# Autodesk Inventor assembly: Prototype Assembly
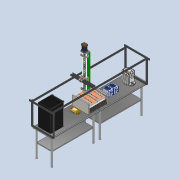
[picture p0: Inventor's stored thumbnail of the model, 180x180]
Saved by Autodesk Inventor 2022 (Build 260153000, 153)
## iProperties
Created: 2021-10-10
Part Number: Prototype Assembly
Document SubType Name: Assembly
Designer: Coy
Author: Coy
## Documents named in this file (14)
- H:\3D Files\Project 3D Models\Breakfast Maker 2000\Assemblys\Prototype Assembly.iam
- H:\3D Files\Project 3D Models\Stock Parts\Workshop\60in Kitchen Prep Table.ipt
- H:\3D Files\Project 3D Models\Stock Parts\Aluminum Extrusion\2040\2040x700 silver profile.ipt
- H:\3D Files\Project 3D Models\Stock Parts\Aluminum Extrusion\2040\2040x1000 silver profile.ipt
- H:\3D Files\Project 3D Models\Stock Parts\Workshop\27in Tall Mini Fridge.ipt
- H:\3D Files\Project 3D Models\Stock Parts\Aluminum Extrusion\2040\2040x800 silver profile.ipt
- H:\3D Files\Project 3D Models\Stock Parts\Workshop\Kureig Assembly.iam
- H:\3D Files\Project 3D Models\Stock Parts\Workshop\Roller hot dogs.ipt
- H:\3D Files\Project 3D Models\Stock Parts\Workshop\TOASTER_BY_TRISTAN_CANNAN.iam
- H:\3D Files\Project 3D Models\Stock Parts\Workshop\waffle_maker.ipt
- H:\3D Files\Project 3D Models\Stock Parts\Linear Actuators\Ball Screw Linear Actuator.iam
- H:\3D Files\Project 3D Models\Stock Parts\Linear Actuators\MGN12C Linear Rail.iam
- H:\3D Files\Downloaded 3D Files\GrabCad Downloads\hiwin-mgn-series-full-2.snapshot.14\PRODUCT_NAME_10.ipt
- H:\3D Files\Project 3D Models\Breakfast Maker 2000\Generic 4x3in Steel Square Tubing.ipt
## Components (40 placed, 13 different names)
1. 60in Kitchen Prep Table:1 — Flush:1, Mate:1, Flush:2, Mate:3, Mate:25, Mate:26, Mate:27, Mate:28
2. 60in Kitchen Prep Table:2 — Flush:1, Mate:1, Flush:2, Mate:2, Flush:3, Flush:5, Mate:20, Flush:36, Mate:24
3. 2040x700 silver profile:1 — Mate:2, Flush:3, Flush:4, Flush:5, Flush:7, Flush:9, Mate:16, Flush:30, Mate:17, Flush:31, Mate:21
4. 2040x700 silver profile:2 — Mate:3, Flush:4, Flush:11, Flush:13, Mate:14, Mate:15, Flush:28, Flush:29
5. 2040x700 silver profile:3 — Flush:13, Flush:27, Mate:14, Flush:28
6. 2040x700 silver profile:4 — Flush:11, Mate:15, Flush:29, Mate:23
7. 2040x700 silver profile:5 — Flush:9, Mate:9, Flush:17, Flush:18, Mate:17, Flush:31
8. 2040x700 silver profile:6 — Flush:7, Mate:8, Flush:15, Flush:16, Mate:16, Flush:30, Mate:22, Flush:38, Flush:39
9. 2040x1000 silver profile:1 — Mate:12, Flush:23, Flush:24
10. 2040x1000 silver profile:2 — Mate:11, Flush:21, Flush:22, Mate:12, Flush:23, Flush:24
11. 2040x1000 silver profile:3 — Mate:8, Flush:15, Flush:16, Mate:10, Flush:19, Flush:20, Mate:29, Flush:42
12. 2040x1000 silver profile:4 — Mate:9, Flush:17, Flush:18, Mate:11, Flush:21, Flush:22
13. 2040x1000 silver profile:5 — Mate:10, Flush:19, Flush:20, Mate:13, Flush:25, Flush:26, Mate:30
14. 2040x1000 silver profile:6 — Mate:13, Flush:25, Flush:26, Flush:27, Flush:41
15. 27in Tall Mini Fridge:1 — Mate:20, Mate:21, Flush:36
16. 2040x800 silver profile:1 — Mate:22, Flush:38, Flush:39, Flush:40
17. 2040x800 silver profile:2 — Mate:23, Flush:40, Flush:41
18. Kureig Assembly:1 [sub-assembly] — Mate:26
19. Roller hot dogs:1 — Mate:25
20. TOASTER_BY_TRISTAN_CANNAN:1 [sub-assembly] — Mate:27
21. waffle_maker:1 — Mate:24
22. TOASTER_BY_TRISTAN_CANNAN:2 [sub-assembly] — Mate:28
23. 2040x700 silver profile:7 — Mate:30, Flush:43, Mate:31, Mate:33, Flush:46, Flush:58
24. 2040x700 silver profile:8 — Mate:29, Flush:42, Flush:43, Mate:31, Mate:32, Flush:45, Mate:34, Flush:47, Mate:35
25. Ball Screw Linear Actuator:1 [sub-assembly] — Mate:49, Flush:72
26. MGN12C Linear Rail:1 [sub-assembly] — Mate:32, Flush:44, Flush:45, Flush:48, Mate:36, Flush:49, Mate:38, Flush:50, Flush:51, Mate:47, Mate:48
27. MGN12C Linear Rail:2 [sub-assembly] — Mate:33, Flush:44, Flush:46, Flush:59, Flush:61, Flush:62, Mate:43, Flush:63, Flush:64
28. PRODUCT_NAME_10:1 — Mate:38, Flush:50, Flush:51, Mate:39, Flush:52, Flush:53
29. PRODUCT_NAME_10:2 — Flush:58, Flush:59, Flush:60, Mate:42
30. PRODUCT_NAME_10:3 — Mate:43, Flush:63, Flush:64, Mate:44, Flush:65, Flush:66
31. PRODUCT_NAME_10:4 — Mate:44, Flush:65, Flush:66, Mate:45, Flush:67, Flush:68
32. PRODUCT_NAME_10:5 — Mate:40, Flush:54, Flush:55, Mate:41, Flush:56, Flush:57
33. PRODUCT_NAME_10:6 — Mate:35, Mate:36, Mate:37, Flush:49
34. PRODUCT_NAME_10:7 — Mate:39, Flush:52, Flush:53, Mate:40, Flush:54, Flush:55
35. PRODUCT_NAME_10:8 — Mate:42, Flush:61, Flush:62
36. PRODUCT_NAME_10:9 — Mate:45, Flush:67, Flush:68, Mate:46, Flush:69, Flush:70
37. PRODUCT_NAME_10:10 — Mate:46, Flush:69, Flush:70
38. PRODUCT_NAME_10:11 — Mate:41, Flush:56, Flush:57
39. PRODUCT_NAME_10:12 — Mate:34, Flush:47, Flush:48, Mate:37, Flush:60
40. Generic 4x3in Steel Square Tubing:1 — Mate:47, Mate:48, Mate:49, Flush:72
## Relationships (104: Flush 61, Mate 43)
- Flush:1: 60in Kitchen Prep Table:1 ↔ 60in Kitchen Prep Table:2
- Mate:1 (1.27 mm): 60in Kitchen Prep Table:1 ↔ 60in Kitchen Prep Table:2
- Flush:2: 60in Kitchen Prep Table:1 ↔ 60in Kitchen Prep Table:2
- Mate:2: 60in Kitchen Prep Table:2 ↔ 2040x700 silver profile:1
- Mate:3: 60in Kitchen Prep Table:1 ↔ 2040x700 silver profile:2
- Flush:3 (-45.2 mm): 60in Kitchen Prep Table:2 ↔ 2040x700 silver profile:1
- Flush:4: 2040x700 silver profile:1 ↔ 2040x700 silver profile:2
- Flush:5: 60in Kitchen Prep Table:2 ↔ 2040x700 silver profile:1
- Flush:7: 2040x700 silver profile:1 ↔ 2040x700 silver profile:6
- Flush:9: 2040x700 silver profile:1 ↔ 2040x700 silver profile:5
- Flush:11: 2040x700 silver profile:2 ↔ 2040x700 silver profile:4
- Flush:13: 2040x700 silver profile:2 ↔ 2040x700 silver profile:3
- Mate:8: 2040x700 silver profile:6 ↔ 2040x1000 silver profile:3
- Flush:15: 2040x700 silver profile:6 ↔ 2040x1000 silver profile:3
- Flush:16: 2040x700 silver profile:6 ↔ 2040x1000 silver profile:3
- Mate:9: 2040x700 silver profile:5 ↔ 2040x1000 silver profile:4
- Flush:17: 2040x700 silver profile:5 ↔ 2040x1000 silver profile:4
- Flush:18: 2040x700 silver profile:5 ↔ 2040x1000 silver profile:4
- Mate:10: 2040x1000 silver profile:3 ↔ 2040x1000 silver profile:5
- Flush:19: 2040x1000 silver profile:3 ↔ 2040x1000 silver profile:5
- Flush:20: 2040x1000 silver profile:3 ↔ 2040x1000 silver profile:5
- Mate:11: 2040x1000 silver profile:2 ↔ 2040x1000 silver profile:4
- Flush:21: 2040x1000 silver profile:2 ↔ 2040x1000 silver profile:4
- Flush:22: 2040x1000 silver profile:2 ↔ 2040x1000 silver profile:4
- Mate:12: 2040x1000 silver profile:1 ↔ 2040x1000 silver profile:2
- Flush:23: 2040x1000 silver profile:1 ↔ 2040x1000 silver profile:2
- Flush:24: 2040x1000 silver profile:1 ↔ 2040x1000 silver profile:2
- Mate:13: 2040x1000 silver profile:5 ↔ 2040x1000 silver profile:6
- Flush:25: 2040x1000 silver profile:5 ↔ 2040x1000 silver profile:6
- Flush:26: 2040x1000 silver profile:5 ↔ 2040x1000 silver profile:6
- Flush:27: 2040x700 silver profile:3 ↔ 2040x1000 silver profile:6
- Mate:14: 2040x700 silver profile:2 ↔ 2040x700 silver profile:3
- Mate:15: 2040x700 silver profile:2 ↔ 2040x700 silver profile:4
- Flush:28: 2040x700 silver profile:2 ↔ 2040x700 silver profile:3
- Flush:29: 2040x700 silver profile:2 ↔ 2040x700 silver profile:4
- Mate:16: 2040x700 silver profile:1 ↔ 2040x700 silver profile:6
- Flush:30: 2040x700 silver profile:1 ↔ 2040x700 silver profile:6
- Mate:17: 2040x700 silver profile:1 ↔ 2040x700 silver profile:5
- Flush:31: 2040x700 silver profile:1 ↔ 2040x700 silver profile:5
- Mate:20 (25.4 mm): 60in Kitchen Prep Table:2 ↔ 27in Tall Mini Fridge:1
- Mate:21 (25.4 mm): 2040x700 silver profile:1 ↔ 27in Tall Mini Fridge:1
- Flush:36 (108.712 mm): 60in Kitchen Prep Table:2 ↔ 27in Tall Mini Fridge:1
- Mate:22: 2040x700 silver profile:6 ↔ 2040x800 silver profile:1
- Flush:38: 2040x700 silver profile:6 ↔ 2040x800 silver profile:1
- Flush:39 (-50 mm): 2040x700 silver profile:6 ↔ 2040x800 silver profile:1
- Mate:23: 2040x700 silver profile:4 ↔ 2040x800 silver profile:2
- Flush:40: 2040x800 silver profile:1 ↔ 2040x800 silver profile:2
- Flush:41: 2040x1000 silver profile:6 ↔ 2040x800 silver profile:2
- Mate:24: 60in Kitchen Prep Table:2 ↔ waffle_maker:1
- Mate:25: 60in Kitchen Prep Table:1 ↔ Roller hot dogs:1
- Mate:26: 60in Kitchen Prep Table:1 ↔ Kureig Assembly:1
- Mate:27: 60in Kitchen Prep Table:1 ↔ TOASTER_BY_TRISTAN_CANNAN:1
- Mate:28: 60in Kitchen Prep Table:1 ↔ TOASTER_BY_TRISTAN_CANNAN:2
- Mate:29 (25.4 mm): 2040x1000 silver profile:3 ↔ 2040x700 silver profile:8
- Flush:42: 2040x1000 silver profile:3 ↔ 2040x700 silver profile:8
- Mate:30 (25.4 mm): 2040x1000 silver profile:5 ↔ 2040x700 silver profile:7
- Flush:43: 2040x700 silver profile:7 ↔ 2040x700 silver profile:8
- Mate:31 (40 mm): 2040x700 silver profile:7 ↔ 2040x700 silver profile:8
- Mate:32: 2040x700 silver profile:8 ↔ MGN12C Linear Rail:1
- Mate:33: 2040x700 silver profile:7 ↔ MGN12C Linear Rail:2
- Flush:44: MGN12C Linear Rail:1 ↔ MGN12C Linear Rail:2
- Flush:45 (4 mm): 2040x700 silver profile:8 ↔ MGN12C Linear Rail:1
- Flush:46 (4 mm): 2040x700 silver profile:7 ↔ MGN12C Linear Rail:2
- Mate:34: 2040x700 silver profile:8 ↔ PRODUCT_NAME_10:12
- Flush:47: 2040x700 silver profile:8 ↔ PRODUCT_NAME_10:12
- Flush:48: MGN12C Linear Rail:1 ↔ PRODUCT_NAME_10:12
- Mate:35: 2040x700 silver profile:8 ↔ PRODUCT_NAME_10:6
- Mate:36: MGN12C Linear Rail:1 ↔ PRODUCT_NAME_10:6
- Mate:37: PRODUCT_NAME_10:6 ↔ PRODUCT_NAME_10:12
- Flush:49: MGN12C Linear Rail:1 ↔ PRODUCT_NAME_10:6
- Mate:38: MGN12C Linear Rail:1 ↔ PRODUCT_NAME_10:1
- Flush:50: MGN12C Linear Rail:1 ↔ PRODUCT_NAME_10:1
- Flush:51: MGN12C Linear Rail:1 ↔ PRODUCT_NAME_10:1
- Mate:39: PRODUCT_NAME_10:1 ↔ PRODUCT_NAME_10:7
- Flush:52: PRODUCT_NAME_10:1 ↔ PRODUCT_NAME_10:7
- Flush:53: PRODUCT_NAME_10:1 ↔ PRODUCT_NAME_10:7
- Mate:40: PRODUCT_NAME_10:5 ↔ PRODUCT_NAME_10:7
- Flush:54: PRODUCT_NAME_10:5 ↔ PRODUCT_NAME_10:7
- Flush:55: PRODUCT_NAME_10:5 ↔ PRODUCT_NAME_10:7
- Mate:41: PRODUCT_NAME_10:5 ↔ PRODUCT_NAME_10:11
- Flush:56: PRODUCT_NAME_10:5 ↔ PRODUCT_NAME_10:11
- Flush:57: PRODUCT_NAME_10:5 ↔ PRODUCT_NAME_10:11
- Flush:58: 2040x700 silver profile:7 ↔ PRODUCT_NAME_10:2
- Flush:59: MGN12C Linear Rail:2 ↔ PRODUCT_NAME_10:2
- Flush:60: PRODUCT_NAME_10:2 ↔ PRODUCT_NAME_10:12
- Mate:42: PRODUCT_NAME_10:2 ↔ PRODUCT_NAME_10:8
- Flush:61: MGN12C Linear Rail:2 ↔ PRODUCT_NAME_10:8
- Flush:62: MGN12C Linear Rail:2 ↔ PRODUCT_NAME_10:8
- Mate:43: MGN12C Linear Rail:2 ↔ PRODUCT_NAME_10:3
- Flush:63: MGN12C Linear Rail:2 ↔ PRODUCT_NAME_10:3
- Flush:64: MGN12C Linear Rail:2 ↔ PRODUCT_NAME_10:3
- Mate:44: PRODUCT_NAME_10:3 ↔ PRODUCT_NAME_10:4
- Flush:65: PRODUCT_NAME_10:3 ↔ PRODUCT_NAME_10:4
- Flush:66: PRODUCT_NAME_10:3 ↔ PRODUCT_NAME_10:4
- Mate:45: PRODUCT_NAME_10:4 ↔ PRODUCT_NAME_10:9
- Flush:67: PRODUCT_NAME_10:4 ↔ PRODUCT_NAME_10:9
- Flush:68: PRODUCT_NAME_10:4 ↔ PRODUCT_NAME_10:9
- Mate:46: PRODUCT_NAME_10:9 ↔ PRODUCT_NAME_10:10
- Flush:69: PRODUCT_NAME_10:9 ↔ PRODUCT_NAME_10:10
- Flush:70: PRODUCT_NAME_10:9 ↔ PRODUCT_NAME_10:10
- Mate:47: MGN12C Linear Rail:1 ↔ Generic 4x3in Steel Square Tubing:1
- Mate:48 (3.5 mm): MGN12C Linear Rail:1 ↔ Generic 4x3in Steel Square Tubing:1
- Mate:49: Ball Screw Linear Actuator:1 ↔ Generic 4x3in Steel Square Tubing:1
- Flush:72 (-50.8 mm): Ball Screw Linear Actuator:1 ↔ Generic 4x3in Steel Square Tubing:1
